# Autodesk Inventor assembly: main body
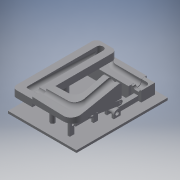
[picture p0: Inventor's stored thumbnail of the model, 180x180]
Saved by Autodesk Inventor 2016 (Build 200138000, 138)
## iProperties
Created: 2018-05-06
Part Number: main body
Material: 一般
Document SubType Name: Assembly
Designer: 黃胤瑋
Author: 黃胤瑋
## Documents named in this file (15)
- C:\Users\黃胤瑋\Desktop\mechanism\second generation\main body.iam
- C:\Users\黃胤瑋\Desktop\mechanism\second generation\實體1.ipt
- C:\Users\黃胤瑋\Desktop\mechanism\second generation\實體2.ipt
- C:\Users\黃胤瑋\Desktop\mechanism\second generation\實體3.ipt
- C:\Users\黃胤瑋\Desktop\mechanism\second generation\實體4.ipt
- C:\Users\黃胤瑋\Desktop\mechanism\second generation\實體5.ipt
- C:\Users\黃胤瑋\Desktop\mechanism\second generation\實體6.ipt
- C:\Users\黃胤瑋\Desktop\mechanism\second generation\實體7.ipt
- C:\Users\黃胤瑋\Desktop\mechanism\second generation\實體8.ipt
- C:\Users\黃胤瑋\Desktop\mechanism\second generation\實體9.ipt
- C:\Users\黃胤瑋\Desktop\mechanism\second generation\02連桿25.ipt
- C:\Users\黃胤瑋\Desktop\mechanism\second generation\03連桿15.ipt
- C:\Users\黃胤瑋\Desktop\mechanism\second generation\馬達.ipt
- C:\Users\黃胤瑋\Desktop\mechanism\second generation\實體10.ipt
- C:\Users\黃胤瑋\Desktop\mechanism\second generation\銷.ipt
## Components (17 placed, 14 different names)
1. 實體1:1
2. 實體2:1 — 貼合:7, 貼合:8
3. 實體3:1
4. 實體4:1
5. 實體5:1
6. 實體6:1 — 貼合:1, 貼合:2, 貼合:3
7. 實體7:1
8. 實體8:1
9. 實體9:1
10. 02連桿25:1 — 貼合:5, 貼合:6, 貼合:9, 貼合:10, 貼合:11, 齊平:1, 貼合:12, 齊平:2
11. 03連桿15:1 — 貼合:4, 貼合:5, 貼合:6
12. 馬達:1 — 貼合:1, 貼合:2, 貼合:3, 貼合:4, 貼合:14, 齊平:4
13. 實體10:1 — 貼合:7, 貼合:8, 貼合:9, 貼合:10, 齊平:3, 貼合:13
14. 銷:1 — 貼合:11, 齊平:1
15. 銷:2 — 貼合:12, 齊平:2
16. 銷:3 — 齊平:3, 貼合:13
17. 銷:4 — 貼合:14, 齊平:4
## Relationships (18: Mate 14, Flush 4)
- 貼合:1 [Mate]: 實體6:1 ↔ 馬達:1
- 貼合:2 [Mate]: 實體6:1 ↔ 馬達:1
- 貼合:3 [Mate]: 實體6:1 ↔ 馬達:1
- 貼合:4 [Mate]: 03連桿15:1 ↔ 馬達:1
- 貼合:5 [Mate]: 02連桿25:1 ↔ 03連桿15:1
- 貼合:6 [Mate]: 02連桿25:1 ↔ 03連桿15:1
- 貼合:7 [Mate]: 實體2:1 ↔ 實體10:1
- 貼合:8 [Mate]: 實體2:1 ↔ 實體10:1
- 貼合:9 [Mate]: 02連桿25:1 ↔ 實體10:1
- 貼合:10 [Mate]: 02連桿25:1 ↔ 實體10:1
- 貼合:11 [Mate]: 02連桿25:1 ↔ 銷:1
- 齊平:1 [Flush]: 02連桿25:1 ↔ 銷:1
- 貼合:12 [Mate]: 02連桿25:1 ↔ 銷:2
- 齊平:2 [Flush]: 02連桿25:1 ↔ 銷:2
- 齊平:3 [Flush]: 實體10:1 ↔ 銷:3
- 貼合:13 [Mate]: 實體10:1 ↔ 銷:3
- 貼合:14 [Mate]: 馬達:1 ↔ 銷:4
- 齊平:4 [Flush]: 馬達:1 ↔ 銷:4
